# Autodesk Inventor assembly: Pedal
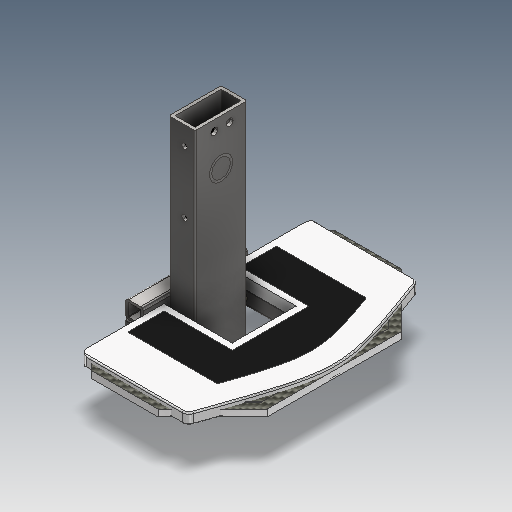
[picture p0: Inventor's stored thumbnail of the model, 512x512]
Saved by Autodesk Inventor 2020 (Build 240168000, 168)
## iProperties
Created: 2019-05-20
Part Number: Pedal
Document SubType Name: Assembly
Designer: chitl
Mass: 738.88 g
Surface Area: 891.506 cm^2
Volume: 163.31 cm^3
Density: 4.5244 g/cm^3
Author: chitl
## Documents named in this file (10)
- C:\Users\chitl\Desktop\OneWheel\Wheel Assembled\Pedal\Pedal.iam
- C:\Users\chitl\Desktop\OneWheel\Wheel Assembled\Pedal\Vertical Tube\Pedal_tube.iam
- C:\Users\chitl\Desktop\OneWheel\Wheel Assembled\Pedal\Footrest\Footrest.iam
- C:\Users\chitl\Desktop\OneWheel\Wheel Assembled\Pedal\Axle\Axle.ipt
- C:\Users\chitl\Desktop\OneWheel\Wheel Assembled\Pedal\Pedal\AIP\FEA\cvs5nll6o.fins
- C:\Users\chitl\Desktop\OneWheel\Wheel Assembled\Pedal\Pedal\AIP\FEA\cvs5nll6o.fsat
- C:\Users\chitl\Desktop\OneWheel\Wheel Assembled\Pedal\Pedal\AIP\FEA\cvs5nll6o.ftes
- C:\Users\chitl\Desktop\OneWheel\Wheel Assembled\Pedal\Pedal\AIP\FEA\cvs5nll6o.fwiz
- C:\Users\chitl\Desktop\OneWheel\Wheel Assembled\Pedal\Pedal\AIP\FEA\cvs5nll9c.fmsh
- C:\Users\chitl\Desktop\OneWheel\Wheel Assembled\Pedal\Pedal\AIP\FEA\cvs5nll9d.fres
## Components (3 placed, 3 different names)
1. Pedal_tube:1 [sub-assembly] — Rigid:1, Angle:1
2. Footrest:1 [sub-assembly] — Insert:1, Angle:1
3. Axle:1 — Rigid:1, Insert:1
## Relationships (3: WeldJoint 1, Insert 1, Angle 1)
- Rigid:1 [WeldJoint] (19.05 mm): Pedal_tube:1 ↔ Axle:1
- Insert:1 (-5.08 mm): Footrest:1 ↔ Axle:1
- Angle:1 (0 deg): Pedal_tube:1 ↔ Footrest:1
## Named parameters: sa_0 = 111206
note: some values were not read from the file. Shown as the stored number, unit unknown: "sa_0".
